# Autodesk Inventor assembly: Nathan_RobotArm_Assembly
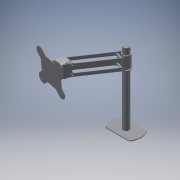
[picture p0: Inventor's stored thumbnail of the model, 180x180]
Saved by Autodesk Inventor 2016 (Build 200138000, 138)
## iProperties
Created: 2017-03-30
Part Number: Nathan_RobotArm_Assembly
Document SubType Name: Assembly
Designer: brandn
Author: brandn
## Documents named in this file (12)
- \\mps\fs\StudentHome\Student2019\brandn\My Documents\Nathan CAD\Nathan_RobotArm\Nathan_RobotArm_Assembly.iam
- \\mps\fs\StudentHome\Student2019\brandn\My Documents\Nathan CAD\Nathan_RobotArm\Nathan_RobotArm_Shaft.ipt
- \\mps\fs\StudentHome\Student2019\brandn\My Documents\Nathan CAD\Nathan_RobotArm\Nathan_RobotArm_TwistPart.ipt
- \\mps\fs\StudentHome\Student2019\brandn\My Documents\Nathan CAD\Nathan_RobotArm\Nathan_RobotArm_Washer.ipt
- \\mps\fs\StudentHome\Student2019\brandn\My Documents\Nathan CAD\Nathan_RobotArm\Nathan_RobotArm_B.ipt
- \\mps\fs\StudentHome\Student2019\brandn\My Documents\Nathan CAD\Nathan_RobotArm\Nathan_RobotArm_Stopper.ipt
- \\mps\fs\StudentHome\Student2019\brandn\My Documents\Nathan CAD\Nathan_RobotArm\Nathan_RobotArm_Base.ipt
- \\mps\fs\StudentHome\Student2019\brandn\My Documents\Nathan CAD\Nathan_RobotArm\Nathan_RobotArm_Arm.ipt
- \\mps\fs\StudentHome\Student2019\brandn\My Documents\Nathan CAD\Nathan_RobotArm\Assembly Twist.iam
- \\mps\fs\StudentHome\Student2019\brandn\My Documents\Nathan CAD\Nathan_RobotArm\Nathan_RobotArm_Bolt3.0.ipt
- \\mps\fs\StudentHome\Student2019\brandn\My Documents\Nathan CAD\Nathan_RobotArm\Swivel.iam
- \\mps\fs\StudentHome\Student2019\brandn\My Documents\Nathan CAD\Nathan_RobotArm\Nathan_RobotArm_WALL.ipt
## Components (18 placed, 11 different names)
1. Nathan_RobotArm_Shaft:1 — Rigid:1, Rigid:4, Rigid:5
2. Nathan_RobotArm_Washer:1 — Rigid:1
3. Nathan_RobotArm_B:1 — Mate:16, Mate:17, Mate:18, Mate:21, Mate:24, Mate:25
4. Nathan_RobotArm_B:2 — Mate:13, Mate:14, Mate:15, Mate:19, Mate:20, Mate:22, Mate:23, Flush:2
5. Nathan_RobotArm_Stopper:1 — Rigid:4
6. Nathan_RobotArm_Base:1 — Rigid:5
7. Nathan_RobotArm_Arm:1 — Mate:6, Mate:7, Mate:15
8. Nathan_RobotArm_Arm:2 — Mate:3, Mate:4, Mate:16, Mate:17
9. Nathan_RobotArm_Arm:3 — Mate:8, Mate:9, Mate:18
10. Nathan_RobotArm_Arm:4 — Mate:1, Mate:2, Mate:13, Mate:14
11. Nathan_RobotArm_TwistPart:2 — Mate:24, Mate:25, Flush:2, Rotational:2
12. Assembly Twist:1 [sub-assembly] — Flush:1, Mate:1, Mate:2, Mate:3, Mate:4, Mate:5, Mate:6, Mate:7, Mate:8, Mate:9, Mate:10, Mate:11
13. Nathan_RobotArm_Bolt3.0:1 — Flush:1
14. Nathan_RobotArm_Bolt3.0:2 — Mate:5, Mate:10, Mate:11
15. Nathan_RobotArm_Bolt3.0:3 — Mate:19, Mate:20, Mate:21
16. Nathan_RobotArm_Bolt3.0:4 — Mate:22, Mate:23
17. Swivel:1 [sub-assembly] — Rotational:2, Mate:26, Mate:27, Mate:28, Mate:29
18. Nathan_RobotArm_WALL:1 — Mate:26, Mate:27, Mate:28, Mate:29
## Relationships (35: Mate 28, WeldJoint 3, RevoluteJoint 2, Flush 2)
- [RevoluteJoint] (-101.6 mm): Nathan_RobotArm_Shaft:1 ↔ Assembly Twist:1
- Rigid:1 [WeldJoint] (-73.66 mm): Nathan_RobotArm_Shaft:1 ↔ Nathan_RobotArm_Washer:1
- Rigid:4 [WeldJoint]: Nathan_RobotArm_Shaft:1 ↔ Nathan_RobotArm_Stopper:1
- Rigid:5 [WeldJoint]: Nathan_RobotArm_Shaft:1 ↔ Nathan_RobotArm_Base:1
- Flush:1: Assembly Twist:1 ↔ Nathan_RobotArm_Bolt3.0:1
- Mate:1: Nathan_RobotArm_Arm:4 ↔ Assembly Twist:1
- Mate:2: Nathan_RobotArm_Arm:4 ↔ Assembly Twist:1
- Mate:3: Nathan_RobotArm_Arm:2 ↔ Assembly Twist:1
- Mate:4: Nathan_RobotArm_Arm:2 ↔ Assembly Twist:1
- Mate:5: Assembly Twist:1 ↔ Nathan_RobotArm_Bolt3.0:2
- Mate:6: Nathan_RobotArm_Arm:1 ↔ Assembly Twist:1
- Mate:7: Nathan_RobotArm_Arm:1 ↔ Assembly Twist:1
- Mate:8: Nathan_RobotArm_Arm:3 ↔ Assembly Twist:1
- Mate:9: Nathan_RobotArm_Arm:3 ↔ Assembly Twist:1
- Mate:10: Assembly Twist:1 ↔ Nathan_RobotArm_Bolt3.0:2
- Mate:11: Assembly Twist:1 ↔ Nathan_RobotArm_Bolt3.0:2
- Mate:13: Nathan_RobotArm_B:2 ↔ Nathan_RobotArm_Arm:4
- Mate:14: Nathan_RobotArm_B:2 ↔ Nathan_RobotArm_Arm:4
- Mate:15: Nathan_RobotArm_B:2 ↔ Nathan_RobotArm_Arm:1
- Mate:16: Nathan_RobotArm_B:1 ↔ Nathan_RobotArm_Arm:2
- Mate:17: Nathan_RobotArm_B:1 ↔ Nathan_RobotArm_Arm:2
- Mate:18: Nathan_RobotArm_B:1 ↔ Nathan_RobotArm_Arm:3
- Mate:19: Nathan_RobotArm_B:2 ↔ Nathan_RobotArm_Bolt3.0:3
- Mate:20: Nathan_RobotArm_B:2 ↔ Nathan_RobotArm_Bolt3.0:3
- Mate:21: Nathan_RobotArm_B:1 ↔ Nathan_RobotArm_Bolt3.0:3
- Mate:22: Nathan_RobotArm_B:2 ↔ Nathan_RobotArm_Bolt3.0:4
- Mate:23: Nathan_RobotArm_B:2 ↔ Nathan_RobotArm_Bolt3.0:4
- Mate:24: Nathan_RobotArm_B:1 ↔ Nathan_RobotArm_TwistPart:2
- Mate:25: Nathan_RobotArm_B:1 ↔ Nathan_RobotArm_TwistPart:2
- Flush:2: Nathan_RobotArm_B:2 ↔ Nathan_RobotArm_TwistPart:2
- Rotational:2 [RevoluteJoint]: Nathan_RobotArm_TwistPart:2 ↔ Swivel:1
- Mate:26: Swivel:1 ↔ Nathan_RobotArm_WALL:1
- Mate:27: Swivel:1 ↔ Nathan_RobotArm_WALL:1
- Mate:28: Swivel:1 ↔ Nathan_RobotArm_WALL:1
- Mate:29: Swivel:1 ↔ Nathan_RobotArm_WALL:1
